# Autodesk Inventor assembly: Microwave Detection Region
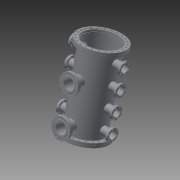
[picture p0: Inventor's stored thumbnail of the model, 180x180]
Saved by Autodesk Inventor 2015 (Build 190159000, 159)
## iProperties
Created: 2014-05-15
Part Number: Microwave Detection Region
Document SubType Name: Assembly
Designer: ijs09
Author: ijs09
## Documents named in this file (5)
- C:\ColdMatter\CADFiles\EDM Machine\Microwave Detection Region\Microwave Detection Region.iam
- C:\ColdMatter\CADFiles\EDM Machine\Microwave Detection Region\Detection Region Vacuum Collar.ipt
- C:\ColdMatter\CADFiles\EDM Machine\Microwave Detection Region\DN200CF.ipt
- C:\ColdMatter\CADFiles\EDM Machine\Microwave Detection Region\DN35CF Counter Bored.ipt
- C:\ColdMatter\CADFiles\EDM Machine\Microwave Detection Region\DN63CF Counter Bored.ipt
## Components (13 placed, 4 different names)
1. Detection Region Vacuum Collar:1 — Mate:24, Mate:25, Mate:26, Mate:27, Mate:33, Mate:34, Mate:35, Mate:36, Mate:37, Mate:38, Mate:39, Mate:40, Mate:41, Mate:42, Mate:43, Mate:44, Rotational:1, Rotational:2, Rotational:3, Rotational:4
2. DN200CF:1 — Mate:24, Mate:25
3. DN200CF:2 — Mate:26, Mate:27
4. DN63CF Counter Bored:1 — Mate:35, Mate:36
5. DN63CF Counter Bored:2 — Mate:33, Mate:34
6. DN35CF Counter Bored:3 — Mate:37, Mate:38
7. DN35CF Counter Bored:4 — Mate:39, Mate:40
8. DN35CF Counter Bored:5 — Mate:41, Mate:42
9. DN35CF Counter Bored:6 — Mate:43, Mate:44
10. DN35CF Counter Bored:7 — Rotational:1
11. DN35CF Counter Bored:8 — Rotational:2
12. DN35CF Counter Bored:9 — Rotational:3
13. DN35CF Counter Bored:10 — Rotational:4
## Relationships (20: Mate 16, RevoluteJoint 4)
- Mate:24: Detection Region Vacuum Collar:1 ↔ DN200CF:1
- Mate:25: Detection Region Vacuum Collar:1 ↔ DN200CF:1
- Mate:26: Detection Region Vacuum Collar:1 ↔ DN200CF:2
- Mate:27: Detection Region Vacuum Collar:1 ↔ DN200CF:2
- Mate:33: Detection Region Vacuum Collar:1 ↔ DN63CF Counter Bored:2
- Mate:34: Detection Region Vacuum Collar:1 ↔ DN63CF Counter Bored:2
- Mate:35: Detection Region Vacuum Collar:1 ↔ DN63CF Counter Bored:1
- Mate:36: Detection Region Vacuum Collar:1 ↔ DN63CF Counter Bored:1
- Mate:37: Detection Region Vacuum Collar:1 ↔ DN35CF Counter Bored:3
- Mate:38: Detection Region Vacuum Collar:1 ↔ DN35CF Counter Bored:3
- Mate:39: Detection Region Vacuum Collar:1 ↔ DN35CF Counter Bored:4
- Mate:40: Detection Region Vacuum Collar:1 ↔ DN35CF Counter Bored:4
- Mate:41: Detection Region Vacuum Collar:1 ↔ DN35CF Counter Bored:5
- Mate:42: Detection Region Vacuum Collar:1 ↔ DN35CF Counter Bored:5
- Mate:43: Detection Region Vacuum Collar:1 ↔ DN35CF Counter Bored:6
- Mate:44: Detection Region Vacuum Collar:1 ↔ DN35CF Counter Bored:6
- Rotational:1 [RevoluteJoint]: Detection Region Vacuum Collar:1 ↔ DN35CF Counter Bored:7
- Rotational:2 [RevoluteJoint]: Detection Region Vacuum Collar:1 ↔ DN35CF Counter Bored:8
- Rotational:3 [RevoluteJoint]: Detection Region Vacuum Collar:1 ↔ DN35CF Counter Bored:9
- Rotational:4 [RevoluteJoint]: Detection Region Vacuum Collar:1 ↔ DN35CF Counter Bored:10
